# Autodesk Inventor assembly: ABD_4mm_set
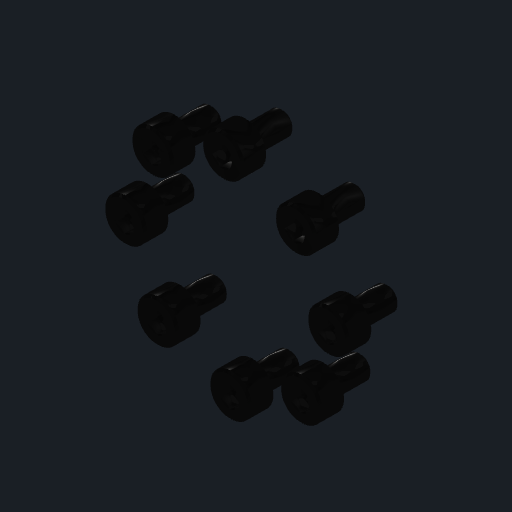
[picture p0: Inventor's stored thumbnail of the model, 512x512]
Saved by Autodesk Inventor 2024.3 (Build 283343000, 343)
## iProperties
Created: 2024-01-28
Part Number: ABD_4mm_set
Document SubType Name: Assembly
Designer: 김대겸
Author: 김대겸
## Documents named in this file (2)
- C:\Users\ASUS\Desktop\test\Screw_Set\ABD_4mm_set.iam
- C:\Users\ASUS\Desktop\test\v1_Frame\MISUMI\CSH-ST-M2_5-4.ipt
## Components (8 placed, 1 different names)
1. CSH-ST-M2_5-4:1
2. CSH-ST-M2_5-4:2
3. CSH-ST-M2_5-4:3
4. CSH-ST-M2_5-4:4
5. CSH-ST-M2_5-4:5
6. CSH-ST-M2_5-4:6
7. CSH-ST-M2_5-4:7
8. CSH-ST-M2_5-4:8
## Relationships (1: Flush 1)
- [Flush]: CSH-ST-M2_5-4:1 ↔ CSH-ST-M2_5-4:8
